# Autodesk Inventor assembly: ParallelMecha_V2_BaseFrame_Item
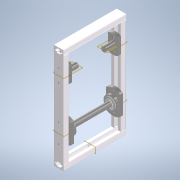
[picture p0: Inventor's stored thumbnail of the model, 180x180]
Saved by Autodesk Inventor 2022 (Build 260153000, 153)
## iProperties
Created: 2022-08-03
Part Number: ParallelMecha_V2_BaseFrame_Item
Document SubType Name: Assembly
Designer: alexw
Author: alexw
## Documents named in this file (10)
- C:\Users\alexw\Documents\Inventor\Projects\03_CurrentProjects\MasterThesis\PSM_V1_Rillenkugellager\ParallelMecha_V2_BaseFrame_Item.iam
- C:\Users\alexw\Documents\Inventor\Projects\03_CurrentProjects\MasterThesis\PSM_V1_Rillenkugellager\Item\item_0026591_profil_5_16x8_5_l_120_details_3.ipt
- C:\Users\alexw\Documents\Inventor\Projects\03_CurrentProjects\MasterThesis\PSM_V1_Rillenkugellager\Item\item_0026591_profil_5_16x8_5_l_200_details_3.ipt
- C:\Users\alexw\Documents\Inventor\Projects\03_CurrentProjects\MasterThesis\PSM_V1_Rillenkugellager\ParallelMecha_V2_BaseFrame_Proximal.ipt
- C:\Users\alexw\Documents\Inventor\Projects\03_CurrentProjects\MasterThesis\PSM_V1_Rillenkugellager\ParallelMecha_DrivenLink_ShaftFixation.ipt
- C:\Users\alexw\Documents\Inventor\Projects\03_CurrentProjects\MasterThesis\PSM_V1_Rillenkugellager\Maschinenbauteil\SKF_W 628_8 R-2RS1\SKF_W 628_8 R-2RS1.iam
- C:\Users\alexw\Documents\Inventor\Projects\03_CurrentProjects\MasterThesis\PSM_V1_Rillenkugellager\ParallelMecha_DrivenShaft.ipt
- C:\Users\alexw\Documents\Inventor\Projects\03_CurrentProjects\MasterThesis\PSM_V1_Rillenkugellager\ParallelMecha_Supportlink_BottomShaft.ipt
- C:\Users\alexw\Documents\Inventor\Projects\03_CurrentProjects\MasterThesis\PSM_V1_Rillenkugellager\Maschinenbauteil\circlips_din471_8_0_8.ipt
- C:\Users\alexw\Documents\Inventor\Projects\03_CurrentProjects\MasterThesis\PSM_V1_Rillenkugellager\Maschinenbauteil\din_988_8_x_14_x_0_10.ipt
## Components (15 placed, 9 different names)
1. ParallelMecha_V2_BaseFrame_Proximal:1 — Fluchtend:1, Fluchtend:2, Passend:31, Passend:32, Fluchtend:3, Fluchtend:4, Passend:36, Fluchtend:5, Fluchtend:6
2. ParallelMecha_DrivenLink_ShaftFixation:1 — Passend:29, Passend:30, Passend:38, Passend:39, Passend:40
3. ParallelMecha_DrivenLink_ShaftFixation:2 — Passend:27, Passend:28, Passend:33, Passend:34, Passend:35
4. SKF_W 628_8 R-2RS1:1 [sub-assembly] — Passend:27, Passend:28, Fluchtend:9, Passend:49
5. SKF_W 628_8 R-2RS1:2 [sub-assembly] — Passend:29, Passend:30, Passend:41, Passend:53
6. item_0026591_profil_5_16x8_5_l_120_details_3:1 — Fluchtend:7, Fluchtend:8, Passend:37
7. item_0026591_profil_5_16x8_5_l_200_details_3:1 — Passend:36, Fluchtend:5, Fluchtend:6, Fluchtend:8, Passend:37, Passend:38, Passend:39, Passend:40, Passend:42, Passend:43, Passend:44
8. item_0026591_profil_5_16x8_5_l_200_details_3:2 — Passend:32, Fluchtend:3, Fluchtend:4, Passend:33, Passend:34, Passend:35, Fluchtend:7, Passend:45, Passend:46, Passend:47
9. ParallelMecha_DrivenShaft:1 — Passend:41, Fluchtend:9, Passend:48, Passend:50, Passend:52, Passend:54
10. ParallelMecha_Supportlink_BottomShaft:1 — Passend:42, Passend:43, Passend:44
11. ParallelMecha_Supportlink_BottomShaft:2 — Passend:45, Passend:46, Passend:47
12. circlips_din471_8_0_8:1 — Passend:50, Passend:51
13. circlips_din471_8_0_8:2 — Passend:54, Passend:55
14. din_988_8_x_14_x_0_10:1 — Passend:52, Passend:53, Passend:55
15. din_988_8_x_14_x_0_10:2 — Passend:48, Passend:49, Passend:51
## Relationships (38: Mate 29, Flush 9)
- Passend:27 [Mate]: ParallelMecha_DrivenLink_ShaftFixation:2 ↔ SKF_W 628_8 R-2RS1:1
- Passend:28 [Mate]: ParallelMecha_DrivenLink_ShaftFixation:2 ↔ SKF_W 628_8 R-2RS1:1
- Passend:29 [Mate]: ParallelMecha_DrivenLink_ShaftFixation:1 ↔ SKF_W 628_8 R-2RS1:2
- Passend:30 [Mate]: ParallelMecha_DrivenLink_ShaftFixation:1 ↔ SKF_W 628_8 R-2RS1:2
- Fluchtend:1 [Flush]: ParallelMecha_V2_BaseFrame_Proximal:1
- Fluchtend:2 [Flush]: ParallelMecha_V2_BaseFrame_Proximal:1
- Passend:31 [Mate]: ParallelMecha_V2_BaseFrame_Proximal:1
- Passend:32 [Mate]: ParallelMecha_V2_BaseFrame_Proximal:1 ↔ item_0026591_profil_5_16x8_5_l_200_details_3:2
- Fluchtend:3 [Flush]: ParallelMecha_V2_BaseFrame_Proximal:1 ↔ item_0026591_profil_5_16x8_5_l_200_details_3:2
- Fluchtend:4 [Flush]: ParallelMecha_V2_BaseFrame_Proximal:1 ↔ item_0026591_profil_5_16x8_5_l_200_details_3:2
- Passend:33 [Mate]: ParallelMecha_DrivenLink_ShaftFixation:2 ↔ item_0026591_profil_5_16x8_5_l_200_details_3:2
- Passend:34 [Mate]: ParallelMecha_DrivenLink_ShaftFixation:2 ↔ item_0026591_profil_5_16x8_5_l_200_details_3:2
- Passend:35 [Mate]: ParallelMecha_DrivenLink_ShaftFixation:2 ↔ item_0026591_profil_5_16x8_5_l_200_details_3:2
- Passend:36 [Mate]: ParallelMecha_V2_BaseFrame_Proximal:1 ↔ item_0026591_profil_5_16x8_5_l_200_details_3:1
- Fluchtend:5 [Flush]: ParallelMecha_V2_BaseFrame_Proximal:1 ↔ item_0026591_profil_5_16x8_5_l_200_details_3:1
- Fluchtend:6 [Flush]: ParallelMecha_V2_BaseFrame_Proximal:1 ↔ item_0026591_profil_5_16x8_5_l_200_details_3:1
- Fluchtend:7 [Flush]: item_0026591_profil_5_16x8_5_l_120_details_3:1 ↔ item_0026591_profil_5_16x8_5_l_200_details_3:2
- Fluchtend:8 [Flush]: item_0026591_profil_5_16x8_5_l_120_details_3:1 ↔ item_0026591_profil_5_16x8_5_l_200_details_3:1
- Passend:37 [Mate]: item_0026591_profil_5_16x8_5_l_120_details_3:1 ↔ item_0026591_profil_5_16x8_5_l_200_details_3:1
- Passend:38 [Mate]: ParallelMecha_DrivenLink_ShaftFixation:1 ↔ item_0026591_profil_5_16x8_5_l_200_details_3:1
- Passend:39 [Mate]: ParallelMecha_DrivenLink_ShaftFixation:1 ↔ item_0026591_profil_5_16x8_5_l_200_details_3:1
- Passend:40 [Mate]: ParallelMecha_DrivenLink_ShaftFixation:1 ↔ item_0026591_profil_5_16x8_5_l_200_details_3:1
- Passend:41 [Mate]: SKF_W 628_8 R-2RS1:2 ↔ ParallelMecha_DrivenShaft:1
- Fluchtend:9 [Flush]: SKF_W 628_8 R-2RS1:1 ↔ ParallelMecha_DrivenShaft:1
- Passend:42 [Mate]: item_0026591_profil_5_16x8_5_l_200_details_3:1 ↔ ParallelMecha_Supportlink_BottomShaft:1
- Passend:43 [Mate]: item_0026591_profil_5_16x8_5_l_200_details_3:1 ↔ ParallelMecha_Supportlink_BottomShaft:1
- Passend:44 [Mate]: item_0026591_profil_5_16x8_5_l_200_details_3:1 ↔ ParallelMecha_Supportlink_BottomShaft:1
- Passend:45 [Mate]: item_0026591_profil_5_16x8_5_l_200_details_3:2 ↔ ParallelMecha_Supportlink_BottomShaft:2
- Passend:46 [Mate]: item_0026591_profil_5_16x8_5_l_200_details_3:2 ↔ ParallelMecha_Supportlink_BottomShaft:2
- Passend:47 [Mate]: item_0026591_profil_5_16x8_5_l_200_details_3:2 ↔ ParallelMecha_Supportlink_BottomShaft:2
- Passend:48 [Mate]: ParallelMecha_DrivenShaft:1 ↔ din_988_8_x_14_x_0_10:2
- Passend:49 [Mate]: SKF_W 628_8 R-2RS1:1 ↔ din_988_8_x_14_x_0_10:2
- Passend:50 [Mate]: ParallelMecha_DrivenShaft:1 ↔ circlips_din471_8_0_8:1
- Passend:51 [Mate]: circlips_din471_8_0_8:1 ↔ din_988_8_x_14_x_0_10:2
- Passend:52 [Mate]: ParallelMecha_DrivenShaft:1 ↔ din_988_8_x_14_x_0_10:1
- Passend:53 [Mate]: SKF_W 628_8 R-2RS1:2 ↔ din_988_8_x_14_x_0_10:1
- Passend:54 [Mate]: ParallelMecha_DrivenShaft:1 ↔ circlips_din471_8_0_8:2
- Passend:55 [Mate]: circlips_din471_8_0_8:2 ↔ din_988_8_x_14_x_0_10:1
